# Autodesk Inventor assembly: ASY DMF 010 cap v2.1
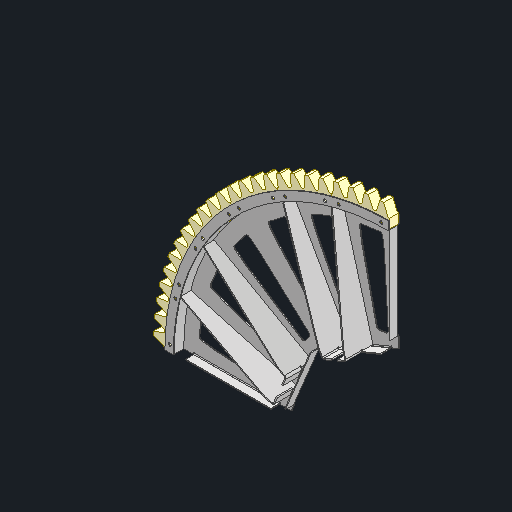
[picture p0: Inventor's stored thumbnail of the model, 512x512]
Saved by Autodesk Inventor 2026.2 (Build 302298000, 298)
## iProperties
Created: 2024-04-30
Part Number: ASY DMF 010 cap v2.1
Document SubType Name: Assembly
Designer: admin
Author: admin
## Documents named in this file (6)
- C:\Users\admin\Documents\Inventor\DMF-Disk-Micro-Filter\Барабан v2.1\ASY DMF 010 cap v2.1.iam
- C:\Users\admin\Documents\Inventor\DMF-Disk-Micro-Filter\Барабан v2.1\DMF 2.1 01 43 Gear rim 3.ipt
- C:\Users\admin\Documents\Inventor\DMF-Disk-Micro-Filter\Барабан v2.1\DMF 2.1 01 44 Gear rim 4.ipt
- C:\Users\admin\Documents\Inventor\DMF-Disk-Micro-Filter\шестерни 06.09.2025\DMF sector big gear 2.1.ipt
- C:\Users\admin\Documents\Inventor\DMF-Disk-Micro-Filter\Барабан v2.1\DMF 2.1 Пластина паза большая.ipt
- C:\Users\admin\Documents\Inventor\DMF-Disk-Micro-Filter\Барабан v2.1\DMF 2.1 01 43 Gear rim 3_CPY.ipt
## Components (13 placed, 6 different names)
1. DMF 2.1 01 43 Gear rim 3.ipt:2 — Flush:2, Flush:1, Flush:3, Mate:1, Mate:2, Mate:3, Mate:4, Flush:4, Flush:5, Flush:6, Flush:7
2. DMF 2.1 Пластина паза большая:1 — Mate:1, Flush:4
3. DMF 2.1 01 44 Gear rim 4.ipt:1 — Rigid:8
4. DMF sector big gear 2.1:6
5. DMF sector big gear 2.1:5
6. DMF sector big gear 2.1:4
7. DMF sector big gear 2.1:3
8. DMF sector big gear 2.1:2
9. DMF sector big gear 2.1.ipt:1
10. DMF 2.1 Пластина паза большая:2 — Mate:2, Flush:5
11. DMF 2.1 Пластина паза большая:3 — Mate:3, Flush:7
12. DMF 2.1 Пластина паза большая:4 — Mate:4, Flush:6
13. DMF 2.1 01 43 Gear rim 3_CPY:1 — Rigid:8
## Relationships (19: WeldJoint 8, Flush 7, Mate 4)
- [WeldJoint]: DMF sector big gear 2.1:2 ↔ DMF sector big gear 2.1.ipt:1
- [WeldJoint]: DMF sector big gear 2.1:3 ↔ DMF sector big gear 2.1:2
- [WeldJoint]: DMF sector big gear 2.1:4 ↔ DMF sector big gear 2.1:3
- [WeldJoint]: DMF sector big gear 2.1:5 ↔ DMF sector big gear 2.1:4
- [WeldJoint]: DMF sector big gear 2.1:6 ↔ DMF sector big gear 2.1:5
- [WeldJoint]: DMF 2.1 01 43 Gear rim 3.ipt:2 ↔ DMF sector big gear 2.1.ipt:1
- [WeldJoint]: DMF 2.1 01 43 Gear rim 3.ipt:2 ↔ DMF 2.1 01 44 Gear rim 4.ipt:1
- Flush:2: DMF 2.1 01 43 Gear rim 3.ipt:2
- Flush:1: DMF 2.1 01 43 Gear rim 3.ipt:2
- Flush:3: DMF 2.1 01 43 Gear rim 3.ipt:2
- Mate:1: DMF 2.1 01 43 Gear rim 3.ipt:2 ↔ DMF 2.1 Пластина паза большая:1
- Mate:2: DMF 2.1 01 43 Gear rim 3.ipt:2 ↔ DMF 2.1 Пластина паза большая:2
- Mate:3: DMF 2.1 01 43 Gear rim 3.ipt:2 ↔ DMF 2.1 Пластина паза большая:3
- Mate:4: DMF 2.1 01 43 Gear rim 3.ipt:2 ↔ DMF 2.1 Пластина паза большая:4
- Flush:4: DMF 2.1 01 43 Gear rim 3.ipt:2 ↔ DMF 2.1 Пластина паза большая:1
- Flush:5: DMF 2.1 01 43 Gear rim 3.ipt:2 ↔ DMF 2.1 Пластина паза большая:2
- Flush:6: DMF 2.1 01 43 Gear rim 3.ipt:2 ↔ DMF 2.1 Пластина паза большая:4
- Flush:7: DMF 2.1 01 43 Gear rim 3.ipt:2 ↔ DMF 2.1 Пластина паза большая:3
- Rigid:8 [WeldJoint]: DMF 2.1 01 44 Gear rim 4.ipt:1 ↔ DMF 2.1 01 43 Gear rim 3_CPY:1
